# Autodesk Inventor assembly: gripper
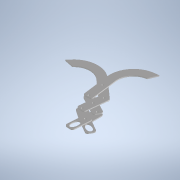
[picture p0: Inventor's stored thumbnail of the model, 180x180]
Saved by Autodesk Inventor 2022 (Build 260153000, 153)
## iProperties
Created: 2022-10-14
Part Number: gripper
Document SubType Name: Assembly
Designer: Usuario
Author: Usuario
## Documents named in this file (4)
- C:\Users\Usuario\Documents\Inventor\Robotica\gripper.iam
- C:\Users\Usuario\Documents\Inventor\Robotica\base.ipt
- C:\Users\Usuario\Documents\Inventor\Robotica\garrita.ipt
- C:\Users\Usuario\Documents\Inventor\Robotica\mitad.ipt
## Components (6 placed, 3 different names)
1. base:1 — Mate:1, Mate:2, Mate:5, Mate:6
2. garrita:1 — Mate:10, Mate:11, Mate:12
3. mitad:1 — Mate:3, Mate:4, Mate:7, Mate:8, Mate:9
4. base:2 — Mate:1, Mate:2, Mate:3, Mate:4
5. garrita:2 — Mate:8, Mate:9, Mate:12
6. mitad:2 — Mate:5, Mate:6, Mate:7, Mate:10, Mate:11
## Relationships (12: Mate 12)
- Mate:1: base:1 ↔ base:2
- Mate:2: base:1 ↔ base:2
- Mate:3: mitad:1 ↔ base:2
- Mate:4: mitad:1 ↔ base:2
- Mate:5: base:1 ↔ mitad:2
- Mate:6: base:1 ↔ mitad:2
- Mate:7: mitad:1 ↔ mitad:2
- Mate:8: mitad:1 ↔ garrita:2
- Mate:9: mitad:1 ↔ garrita:2
- Mate:10: garrita:1 ↔ mitad:2
- Mate:11: garrita:1 ↔ mitad:2
- Mate:12: garrita:1 ↔ garrita:2
